# Autodesk Inventor assembly: flow meter solenoid asm
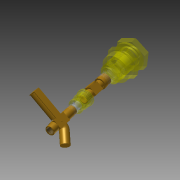
[picture p0: Inventor's stored thumbnail of the model, 180x180]
Saved by Autodesk Inventor 2011 (Build 150239000, 239)
## iProperties
Created: 2013-11-19
Part Number: flow meter solenoid asm
Document SubType Name: Assembly
Designer: Devon
Author: Devon
## Documents named in this file (7)
- C:\Users\Devon\Dropbox\ELEC 4497 - Senior Design\Design\flow\flow meter solenoid asm.iam
- C:\Users\Devon\Dropbox\ELEC 4497 - Senior Design\Design\flow\Imported Components\.5-.375in coupling\.5-.375in coupling.ipt
- C:\Users\Devon\Dropbox\ELEC 4497 - Senior Design\Design\flow\Imported Components\.375 nipple\.375 nipple.ipt
- C:\Users\Devon\Dropbox\ELEC 4497 - Senior Design\Design\flow\half inch flow valve.ipt
- C:\Users\Devon\Dropbox\ELEC 4497 - Senior Design\Design\flow\solenoid valve.ipt
- C:\Users\Devon\Dropbox\ELEC 4497 - Senior Design\Design\flow\Imported Components\.5in nipple\.5in nipple.ipt
- C:\Users\Devon\Dropbox\ELEC 4497 - Senior Design\Design\flow\Imported Components\36895K161\36895K161.ipt
## Components (6 placed, 6 different names)
1. half inch flow valve:1 — Insert:2, Insert:3
2. solenoid valve:1 — Insert:5
3. .375 nipple:1 — Insert:4, Insert:5
4. .5-.375in coupling:1 — Insert:3, Insert:4
5. .5in nipple:1 — Insert:2, Insert:6
6. 36895K161:1 — Insert:6
## Relationships (5: Insert 5)
- Insert:2 (-9.525 mm): half inch flow valve:1 ↔ .5in nipple:1
- Insert:3 (3.175 mm): half inch flow valve:1 ↔ .5-.375in coupling:1
- Insert:4 (3.175 mm): .375 nipple:1 ↔ .5-.375in coupling:1
- Insert:5 (-9.525 mm): solenoid valve:1 ↔ .375 nipple:1
- Insert:6 (9.525 mm): .5in nipple:1 ↔ 36895K161:1
